# Autodesk Inventor assembly: xy_assembly
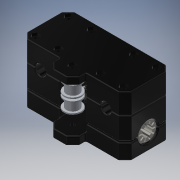
[picture p0: Inventor's stored thumbnail of the model, 180x180]
Saved by Autodesk Inventor 2018 (Build 220112000, 112)
## iProperties
Created: 2018-06-03
Part Number: xy_assembly
Document SubType Name: Assembly
Designer: Z. Deniz
Author: Z. Deniz
## Documents named in this file (6)
- C:\Users\zdeni\Desktop\3d\Yeni klasör\xy_assembly.iam
- C:\Users\zdeni\Desktop\3d\Yeni klasör\xy_joint_top.ipt
- C:\Users\zdeni\Desktop\3d\Yeni klasör\123RJ4JP_01_08_1.ipt
- C:\Users\zdeni\Desktop\3d\Yeni klasör\xy_joint_mid.ipt
- C:\Users\zdeni\Desktop\3d\Yeni klasör\xy_joint_bottom.ipt
- C:\Users\zdeni\Desktop\3d\Yeni klasör\02131021795.ipt
## Components (8 placed, 5 different names)
1. xy_joint_top:1 — Tangent:1, Mate:1, Mate:2, Tangent:2, Flush:1, Flush:2, Flush:3, Flush:4, Flush:7, Insert:2
2. 123RJ4JP_01_08_1:1 — Mate:2, Tangent:2, Mate:4
3. 123RJ4JP_01_08_1:2 — Tangent:1, Mate:1, Mate:3
4. xy_joint_mid:1 — Flush:1, Mate:3, Flush:2, Mate:5, Flush:5, Flush:6, Flush:7, Flush:8
5. xy_joint_mid:2 — Mate:4, Flush:3, Flush:4
6. xy_joint_bottom:1 — Mate:5, Flush:5, Flush:6, Insert:1, Flush:8
7. 02131021795:1 — Insert:2
8. 02131021795:2 — Insert:1
## Relationships (17: Flush 8, Mate 5, Tangent 2, Insert 2)
- Tangent:1: xy_joint_top:1 ↔ 123RJ4JP_01_08_1:2
- Mate:1: xy_joint_top:1 ↔ 123RJ4JP_01_08_1:2
- Mate:2: xy_joint_top:1 ↔ 123RJ4JP_01_08_1:1
- Tangent:2: xy_joint_top:1 ↔ 123RJ4JP_01_08_1:1
- Flush:1: xy_joint_top:1 ↔ xy_joint_mid:1
- Mate:3: 123RJ4JP_01_08_1:2 ↔ xy_joint_mid:1
- Flush:2: xy_joint_top:1 ↔ xy_joint_mid:1
- Mate:4: 123RJ4JP_01_08_1:1 ↔ xy_joint_mid:2
- Flush:3: xy_joint_top:1 ↔ xy_joint_mid:2
- Flush:4: xy_joint_top:1 ↔ xy_joint_mid:2
- Mate:5: xy_joint_mid:1 ↔ xy_joint_bottom:1
- Flush:5: xy_joint_mid:1 ↔ xy_joint_bottom:1
- Flush:6: xy_joint_mid:1 ↔ xy_joint_bottom:1
- Insert:1 (3.049 mm): xy_joint_bottom:1 ↔ 02131021795:2
- Flush:7: xy_joint_top:1 ↔ xy_joint_mid:1
- Flush:8: xy_joint_mid:1 ↔ xy_joint_bottom:1
- Insert:2 (-11.424 mm): xy_joint_top:1 ↔ 02131021795:1
